# Autodesk Inventor assembly: Roller Piston 4 (.5 and 1 in Stroke, 9-16 in Bore)
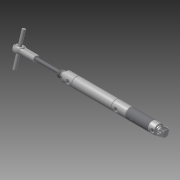
[picture p0: Inventor's stored thumbnail of the model, 180x180]
Saved by Autodesk Inventor 2014 (Build 180170000, 170)
## iProperties
Category: PARTsolutions
Company: BIMBA
Created: 2014-01-20
Part Number: Roller Piston 4 (.5 and 1 in Stroke, 9-16 in Bore)
Catalog Web Link: www.cadenas.de
Description: Original Line Three-Position Cylinders-
Vendor: BIMBA
Document SubType Name: Assembly
Designer: Michael
Manufacturer: BIMBA
PSOL_IDENT_0: {$CADENAS_DATA\23d-libs\bimba\bimba\bimba_imperial\bimba_full_line\original_line_cylinders\three_pos
PSOL_IDENT_1: ition_cylinders\3position_asmtab.prj},283 {VTYP=3D},{STYP=ASSTAB},{NB=020.5/1-DXP(D-12321-A)},{LINA=
PSOL_IDENT_2: 020.5/1-DXP},{NN=Original Line Three-Position Cylinders},{DATE=15.10.2013 05:44:09},{GEOMDATE=27.08.
PSOL_IDENT_3: 2012},{VERSION=},{LINEID=40},{LINESUBID=-1},{WBVAR=STROKEA,STROKEB,MNT,NR,M,NT,EE,EEL,G,K,Q,B,T,W,T1
PSOL_IDENT_4: ,T2,T3,T4,PRC,MB,MN,PB}  {NB=020.5/1-DXP(D-12321-A)},{LINA=020.5/1-DXP},{KT=DUMMY},{PN=020.5/1-DXP},
PSOL_IDENT_5: {PNC=020.5/1-DXP(D-12321-A)},{PNA=(D-12321-A)},{DASH=-},{BORE1=0.56250000},{BORE=9/16\" (02)},{BOREP
PSOL_IDENT_6: N=02},{STROKEA=0.500},{STROKEB=1.000},{STROKEALGA=[0.011:31.989/0.001]},{STROKEALGB=[0.011:31.5/0.00
PSOL_IDENT_7: 1]},{STROKEBMAX=31.5},{STROKE1=0.5},{STROKE2=1.000},{AC=Double Acting},{ACTING=D},{ACTINGALG= 'D' , '
PSOL_IDENT_8: Double Acting' },{ACTINGPN=D},{MNT=XP},{MNTALG= '' , 'Nose Mounting (3P)' , 'XP' , 'Universal Mounti
PSOL_IDENT_9: ng (3P)' },{MNTPN=XP},{TYPE=},{NR=},{NRALG= '' , 'Round (Standard)' , 'NR' , 'Non-Rotating Square' }
PSOL_IDENT_10: ,{NRPN=},{M=},{MALG= '', 'Without Magnet', 'M', 'With Magnet' },{MATR=303 Stainless Steel},{F=},{FAL
PSOL_IDENT_11: G= '', 'Non-Coated (Standard)', 'F', 'Molycoated' },{FPN=},{NT=},{NTPN=},{EE=},{EEL=0.000},{EEMAX=30
PSOL_IDENT_12: .500},{EEALG= '', 'Without Extra Extension', 'EE', 'With Extra Extension' },{EELALG=0},{EEPN=},{EEPN
PSOL_IDENT_13: 1=0.000},{G=},{GPN=},{GPN1=},{K=},{KALG= '', 'Standard' , 'K' , 'Ports Rotated 90deg K' },{KPN=},{Q=
PSOL_IDENT_14: },{QALG= '' , 'N/A' },{QPN=},{B=},{BALG= '', 'Without Bumper' , 'B' , 'With Bumper' },{BPN=},{T=},{T
PSOL_IDENT_15: ALG= '' , 'Standard -20° to 200°F (-29° to 95°C)' , 'N' , 'Low Temperature' , 'V' , 'High Temperatur
PSOL_IDENT_16: e' },{NPN=},{VPN=},{W=},{WALG= '' , 'Without Wiper' , 'W' , 'With Wiper' },{WPN=},{E=},{EALG= '' , '
PSOL_IDENT_17: Standard Seals/Lube' , 'E' , 'Non-Lube Seals/Lube' },{EPN=},{ST=},{STALG= '' , 'Without Switch Track'
PSOL_IDENT_18: , '-' , 'With Switch Track' },{STPALG= '' , 'N/A' },{STPN=},{T1=},{T2=},{T3=},{T4=},{S=},{SALG='','
PSOL_IDENT_19: N/A'},{SPN=},{PRC=},{PRCALG= '' , 'w/out Pivot Rod Clevis' , 'D-850' , 'D-850'},{PRCPN=},{MB=},{MN=}
PSOL_IDENT_20: ,{PB=D-12321-A},{PBALG= '' , 'w/out Pivot Bracket' , 'D-12321-A' , 'D-12321-A' },{PBPN=(D-12321-A)},
PSOL_IDENT_21: {TLEN=2.007},{TEXT=0.133333},{SPACE=0.07619},{FRAC=4.47},{BL=},{BR=},{DWGC=},{PNN=},{MNTRG=},{ACTING
PSOL_IDENT_22: RG=R},{DIMBRL=2.28100000},{DIMBRE=1.65600000},{DIMBBL=1.00000000},{RLB=3.781},{REB=3.156},{BLB=2.500
PSOL_IDENT_23: },{DIMARL=1.85600000},{DIMARE=1.23100000},{DIMABL=0.93800000},{RLA=2.356},{REA=1.731},{BLA=1.438},{D
PSOL_IDENT_24: WGCS=D-68355},{DWGTA=D-75938},{DWGTB=D-7516},{DWGRH=D-15705},{DWGRG=D-26368},{TRANS=0.50000000},{DWG
PSOL_IDENT_25: RCB=D-7508},{DWGRCA=D-9538},{BRL=2.50000000},{BRE=1.57800000},{BBL=1.06200000},{ARL=1.91600000},{ARE=
PSOL_IDENT_26: 0.99400000},{ABL=1.06200000},{T1ALG='','N/A'},{T2ALG='','N/A'},{T3ALG='','N/A'},{T4ALG='','N/A'},{DW
PSOL_IDENT_27: GST=D-74168},{DWGS=},{STL=2.15},{TS=X},{SS=},{AA=4.40},{BA=2.25},{C=0.75},{D=#10-32},{E1=0.38},{E11=
PSOL_IDENT_28: 0.38000000},{E12=0.38000000},{F1=0.06},{G1=N/A},{H=0.50},{I=7/16-20},{J=N/A},{K1=#10-32},{L1=.434/.4
PSOL_IDENT_29: 37},{M1=0.38},{N=0.31},{O=0.62},{AA1=4.12000000},{BA1=2.25000000},{AA1B=4.31000000},{BA1B=2.31000000
PSOL_IDENT_30: },{AA1XP=4.40000000},{BA1XP=2.25000000},{AA1BXP=4.59000000},{BA1BXP=2.31000000},{M11=0.19000000},{M1
PSOL_IDENT_31: 2=0.38000000},{N1=0.50000000},{N2=0.31000000},{O1=0.62000000},{O2=0.62000000},{P=0.25},{Q1=0.19},{R=
PSOL_IDENT_32: 0.16},{P1=0.25000000},{Q11=0.19000000},{R1=0.16},{MBALG= '' , 'w/out Mounting Bracket' , 'F,D-770' ,
PSOL_IDENT_33: 'D-770 (front)', 'R,D-770' , 'D-770 (rear)', '2x,D-770' , 'D-770 (front & rear)' },{MBPN=},{MBP=},{
PSOL_IDENT_34: MNALG= '' , 'w/out Mounting Nut' , 'F,D-154' , 'D-154 (front)', 'R,D-154' , 'D-154 (rear)', '2x,D-15
PSOL_IDENT_35: 4' , 'D-154 (front & rear)' },{MNPN=},{MNP=},{PRCP=},{MBR=},{MBF=},{MNF=},{MNR=},{PBPNALL=D-12321-A}
PSOL_IDENT_36: ,{MBPNALL=D-770},{PRCPNALL=D-850},{FNUTPN=D-154},{RNUTPN=D-154},{ASSOPTACC=T4},{MATALGHTML=<b>Origin
PSOL_IDENT_37: al Line Three Position:</b><dl><dt>Rod:</dt><dd>- 303 Stainless Steel</dd><dt>Bearings:</dt><dd>- Si
PSOL_IDENT_38: ntered Bronze</dd><dt>Body:</dt><dd>- 304 Stainless Steel</dd><dt>End Caps:</dt><dd>- Aluminum</dd><
PSOL_IDENT_39: dt>Seals:</dt><dd>-  Buna N</dd></dl>},{PPATH=three_pos_cylinder_asmtpl.prj}
CNS_NN: Original Line Three-Position Cylinders
CNS_NT: Standard Male Thread
CNS_NB: 020.5/1-DXP(D-12321-A)
CNS_NBSYN: $PNC.
CNS_LINA: 020.5/1-DXP
CNS_PN: 020.5/1-DXP
CNS_PNC: 020.5/1-DXP(D-12321-A)
CNS_PNA: (D-12321-A)
CNS_DASH: -
CNS_BORE1: 0.56250000
CNS_BORE: 9/16" [02]
CNS_BOREPN: 02
CNS_STROKEA: 0.500
CNS_STROKEB: 1.000
CNS_STROKEALGA: [0.011:31.989/0.001]
CNS_STROKEALGB: [0.011:31.5/0.001]
CNS_STROKEBMAX: 31.500
CNS_STROKE1: 0.500
CNS_STROKE2: 1.000
CNS_AC: Double
CNS_ACTING: D
CNS_ACTINGALG: 'D' , 'Double Acting'
CNS_ACTINGPN: D
CNS_MNT: Universal Double End or Rear Pivot [DXP]
CNS_MNTALG: '' , 'Nose Mounting (3P)' , 'XP' , 'Universal Mounting (3P)'
CNS_MNTPN: XP
CNS_NR: Standard Round
CNS_NRALG: '' , 'Round (Standard)' , 'NR' , 'Non-Rotating Square'
CNS_M: Without Magnet Piston
CNS_MALG: '', 'Without Magnet', 'M', 'With Magnet'
CNS_MATR: Stainless Steel
CNS_FALG: '', 'Non-Coated (Standard)', 'F', 'Molycoated'
CNS_EE: Standard Rod Extension
CNS_EEL: 0.000
CNS_EEMAX: 30.500
CNS_EEALG: '', 'Without Extra Extension', 'EE', 'With Extra Extension'
CNS_EELALG: 0
CNS_EEPN1: 0.000
CNS_G: Standard Grease Lube
CNS_K: Standard
CNS_KALG: '', 'Standard' , 'K' , 'Ports Rotated 90deg K'
CNS_Q: N/A
CNS_QALG: '' , 'N/A'
CNS_B: Without Bumpers
CNS_BALG: '', 'Without Bumper' , 'B' , 'With Bumper'
CNS_T: Standard -20° to 200°F (-29° to 95°C)
CNS_TALG: '' , 'Standard -20° to 200°F (-29° to 95°C)' , 'N' , 'Low Temperature' , 'V' , 'High Temperature'
CNS_W: Without Wiper
CNS_WALG: '' , 'Without Wiper' , 'W' , 'With Wiper'
CNS_EALG: '' , 'Standard Seals/Lube' , 'E' , 'Non-Lube Seals/Lube'
CNS_STALG: '' , 'Without Switch Track' , '-' , 'With Switch Track'
CNS_STPALG: '' , 'N/A'
CNS_T1: N/A
CNS_T2: N/A
CNS_T3: N/A
CNS_T4: N/A
CNS_SALG: '','N/A'
CNS_PRC: Without Piston Rod Clevis
CNS_PRCALG: '' , 'w/out Pivot Rod Clevis' , 'D-850' , 'D-850'
CNS_MB: Without Mounting Bracket
CNS_MN: Without Mounting Nut
CNS_PB: D-12321-A
CNS_PBALG: '' , 'w/out Pivot Bracket' , 'D-12321-A' , 'D-12321-A'
CNS_PBPN: (D-12321-A)
CNS_TLEN: 2.007
CNS_TEXT: 0.133
CNS_SPACE: 0.076
CNS_FRAC: 4.470
CNS_ACTINGRG: R
CNS_DIMBRL: 2.28100000
CNS_DIMBRE: 1.65600000
CNS_DIMBBL: 1.00000000
CNS_RLB: 3.781
CNS_REB: 3.156
CNS_BLB: 2.500
CNS_DIMARL: 1.85600000
CNS_DIMARE: 1.23100000
CNS_DIMABL: 0.93800000
CNS_RLA: 2.356
CNS_REA: 1.731
CNS_BLA: 1.438
CNS_DWGCS: D-68355
CNS_DWGTA: D-75938
CNS_DWGTB: D-7516
CNS_DWGRH: D-15705
CNS_DWGRG: D-26368
CNS_TRANS: 0.50000000
CNS_DWGRCB: D-7508
CNS_DWGRCA: D-9538
CNS_BRL: 2.50000000
CNS_BRE: 1.57800000
CNS_BBL: 1.06200000
CNS_ARL: 1.91600000
CNS_ARE: 0.99400000
CNS_ABL: 1.06200000
CNS_T1ALG: '','N/A'
CNS_T2ALG: '','N/A'
CNS_T3ALG: '','N/A'
CNS_T4ALG: '','N/A'
CNS_DWGST: D-74168
CNS_STL: 2.150
CNS_TS: X
CNS_AA: 4.40
CNS_BA: 2.25
CNS_C: 0.75
CNS_D: #10-32
CNS_E1: 0.38
CNS_E11: 0.38000000
CNS_E12: 0.38000000
CNS_F1: 0.06
CNS_G1: N/A
CNS_H: 0.50
CNS_I: 7/16-20
CNS_J: N/A
CNS_K1: #10-32
CNS_L1: .434/.437
CNS_M1: 0.38
CNS_N: 0.31
CNS_O: 0.62
CNS_AA1: 4.12000000
CNS_BA1: 2.25000000
CNS_AA1B: 4.31000000
CNS_BA1B: 2.31000000
CNS_AA1XP: 4.40000000
CNS_BA1XP: 2.25000000
CNS_AA1BXP: 4.59000000
CNS_BA1BXP: 2.31000000
CNS_M11: 0.19000000
CNS_M12: 0.38000000
CNS_N1: 0.50000000
CNS_N2: 0.31000000
CNS_O1: 0.62000000
CNS_O2: 0.62000000
CNS_P: 0.25
CNS_Q1: 0.19
CNS_R: 0.16
CNS_P1: 0.25000000
CNS_Q11: 0.19000000
CNS_R1: 0.16
CNS_MBALG: '' , 'w/out Mounting Bracket' , 'F,D-770' , 'D-770 (front)', 'R,D-770' , 'D-770 (rear)', '2x,D-770' , 'D-770 (front & rear)'
CNS_MNALG: '' , 'w/out Mounting Nut' , 'F,D-154' , 'D-154 (front)', 'R,D-154' , 'D-154 (rear)', '2x,D-154' , 'D-154 (front & rear)'
CNS_PBPNALL: D-12321-A
CNS_MBPNALL: D-770
CNS_PRCPNALL: D-850
CNS_FNUTPN: D-154
CNS_RNUTPN: D-154
CNS_ASSOPTACC: T4
CNS_MATALGHTML: <b>Original Line Three Position:</b><dl><dt>Rod:</dt><dd>- 303 Stainless Steel</dd><dt>Bearings:</dt><dd>- Sintered Bronze</dd><dt>Body:</dt><dd>- 304 Stainless Steel</dd><dt>End Caps:</dt><dd>- Aluminum</dd><dt>Seals:</dt><dd>-  Buna N</dd></dl>
CNS_PPATH: three_pos_cylinder_asmtpl.prj
SUPPLIER: BIMBA
ARTICLENO: 020.5/1-DXP(D-12321-A)
BOMINFO: 020.5/1-DXP
CREATOR: CADENAS GmbH
Title: 020.5/1-DXP
Author: Cadenas PARTsolutions
## Documents named in this file (15)
- C:\Users\Michael\Documents\GitHub\2014buildCAD\Duluth Collector\Roller Piston 4 (.5 and 1 in Stroke, 9-16 in Bore).iam
- C:\Users\Michael\Documents\GitHub\2014buildCAD\New Collector\020_5_1-DXP(D-12321-A)0_dummy.ipt
- C:\Users\Michael\Documents\GitHub\2014buildCAD\New Collector\D-68355-XP--0.ipt
- C:\Users\Michael\Documents\GitHub\2014buildCAD\New Collector\D-75938XP-1_438.ipt
- C:\Users\Michael\Documents\GitHub\2014buildCAD\New Collector\D-15705rear_head.ipt
- C:\Users\Michael\Documents\GitHub\2014buildCAD\New Collector\D-8597.ipt
- C:\Users\Michael\Documents\GitHub\2014buildCAD\New Collector\D-12321-A-dummy.ipt
- C:\Users\Michael\Documents\GitHub\2014buildCAD\New Collector\D-9769-clevis_pin.ipt
- C:\Users\Michael\Documents\GitHub\2014buildCAD\New Collector\D-9770-rr.ipt
- C:\Users\Michael\Documents\GitHub\2014buildCAD\New Collector\D-7516XP-2_5.ipt
- C:\Users\Michael\Documents\GitHub\2014buildCAD\New Collector\D-26368----0_5_rod_guide_cyl.ipt
- C:\Users\Michael\Documents\GitHub\2014buildCAD\New Collector\D-75080_5-1XP-3_781-3pos.ipt
- C:\Users\Michael\Documents\GitHub\2014buildCAD\New Collector\D-95380_5-1XP-2_356-3pos.ipt
- C:\Users\Michael\Documents\GitHub\2014buildCAD\New Collector\Axle 0.190 in 3 in length.ipt
- C:\Users\Michael\Documents\GitHub\2014buildCAD\New Collector\Rod End (McMaster Part #6498K592).ipt
## Components (15 placed, 14 different names)
1. 020_5_1-DXP(D-12321-A)0_dummy:1 — dummy_XY@1 <-> centar_XY@2, dummy_Z@1 <-> centar_Z@2, dummy_YZ@1 <-> centar_YZ@2
2. D-68355-XP--0:1 — dummy_XY@1 <-> centar_XY@2, dummy_Z@1 <-> centar_Z@2, dummy_YZ@1 <-> centar_YZ@2, to_cyl_A_XY@2 <-> tube2_XY@3, to_cyl_A_Z@2 <-> tube2_Z@3, to_cyl_A_YZ@2 <-> tube2_YZ@3, to_cyl_B_XY@2 <-> tube1_XY@12, to_cyl_B_Z@2 <-> tube1_Z@12, to_cyl_B_YZ@2 <-> tube1_YZ@12, to_rod_A_XY@2 <-> to_rod_guide_XY@15, to_rod_A_Z@2 <-> to_rod_guide_Z@15
3. D-75938XP-1_438:1 — to_cyl_A_XY@2 <-> tube2_XY@3, to_cyl_A_Z@2 <-> tube2_Z@3, to_cyl_A_YZ@2 <-> tube2_YZ@3, tube1_XY@3 <-> rear_head_XY@4, tube1_Z@3 <-> rear_head_Z@4, tube1_YZ@3 <-> rear_head_YZ@4
4. D-15705rear_head:1 — tube1_XY@3 <-> rear_head_XY@4, tube1_Z@3 <-> rear_head_Z@4, tube1_YZ@3 <-> rear_head_YZ@4, to_bushing_XY@4 <-> bushing_XY@5, to_bushing_Z@4 <-> bushing_Z@5, to_bushing_YZ@4 <-> bushing_YZ@5, to_pivot_bracket_XY@4 <-> to_cyl_XY@6, to_pivot_bracket_Z@4 <-> to_cyl_Z@6, Mate:33
5. D-8597:1 — to_bushing_XY@4 <-> bushing_XY@5, to_bushing_Z@4 <-> bushing_Z@5, to_bushing_YZ@4 <-> bushing_YZ@5, Mate:32
6. D-12321-A-dummy:1 — to_pivot_bracket_XY@4 <-> to_cyl_XY@6, to_pivot_bracket_Z@4 <-> to_cyl_Z@6
7. D-9769-clevis_pin:1 — rr1_XY@9 <-> rr_XY@10, rr1_Z@9 <-> rr_Z@10, rr1_YZ@9 <-> rr_YZ@10, rr2_XY@9 <-> rr_XY@11, rr2_Z@9 <-> rr_Z@11, rr2_YZ@9 <-> rr_YZ@11, Mate:32
8. D-9770-rr:1 — rr1_XY@9 <-> rr_XY@10, rr1_Z@9 <-> rr_Z@10, rr1_YZ@9 <-> rr_YZ@10, Mate:33
9. D-9770-rr:2 — rr2_XY@9 <-> rr_XY@11, rr2_Z@9 <-> rr_Z@11, rr2_YZ@9 <-> rr_YZ@11
10. D-7516XP-2_5:1 — to_cyl_B_XY@2 <-> tube1_XY@12, to_cyl_B_Z@2 <-> tube1_Z@12, to_cyl_B_YZ@2 <-> tube1_YZ@12, tube2_XY@12 <-> to_tube_XY@13, tube2_Z@12 <-> to_tube_Z@13, tube2_YZ@12 <-> to_tube_YZ@13
11. D-26368----0_5_rod_guide_cyl:1 — tube2_XY@12 <-> to_tube_XY@13, tube2_Z@12 <-> to_tube_Z@13, tube2_YZ@12 <-> to_tube_YZ@13, to_rod_XY@13 <-> to_rod_guide_XY@14, to_rod_Z@13 <-> to_rod_guide_Z@14
12. D-75080_5-1XP-3_781-3pos:1 — to_rod_XY@13 <-> to_rod_guide_XY@14, to_rod_Z@13 <-> to_rod_guide_Z@14, Mate:24, Mate:30
13. D-95380_5-1XP-2_356-3pos:1 — to_rod_A_XY@2 <-> to_rod_guide_XY@15, to_rod_A_Z@2 <-> to_rod_guide_Z@15
14. Axle 0.190 in 3 in length:1 — Mate:26, Flush:6
15. Rod End (McMaster Part #6498K592):1 — Mate:24, Mate:26, Flush:6, Mate:30
## Relationships (36: Mate 24, Angle 8, Flush 4)
- dummy_XY@1 <-> centar_XY@2 [Mate]: 020_5_1-DXP(D-12321-A)0_dummy:1 ↔ D-68355-XP--0:1
- dummy_Z@1 <-> centar_Z@2 [Mate]: 020_5_1-DXP(D-12321-A)0_dummy:1 ↔ D-68355-XP--0:1
- dummy_YZ@1 <-> centar_YZ@2 [Angle] (-90 deg): 020_5_1-DXP(D-12321-A)0_dummy:1 ↔ D-68355-XP--0:1
- to_cyl_A_XY@2 <-> tube2_XY@3 [Flush]: D-68355-XP--0:1 ↔ D-75938XP-1_438:1
- to_cyl_A_Z@2 <-> tube2_Z@3 [Mate]: D-68355-XP--0:1 ↔ D-75938XP-1_438:1
- to_cyl_A_YZ@2 <-> tube2_YZ@3 [Angle] (0 deg): D-68355-XP--0:1 ↔ D-75938XP-1_438:1
- tube1_XY@3 <-> rear_head_XY@4 [Mate]: D-75938XP-1_438:1 ↔ D-15705rear_head:1
- tube1_Z@3 <-> rear_head_Z@4 [Mate]: D-75938XP-1_438:1 ↔ D-15705rear_head:1
- tube1_YZ@3 <-> rear_head_YZ@4 [Angle] (90 deg): D-75938XP-1_438:1 ↔ D-15705rear_head:1
- to_bushing_XY@4 <-> bushing_XY@5 [Mate]: D-15705rear_head:1 ↔ D-8597:1
- to_bushing_Z@4 <-> bushing_Z@5 [Mate]: D-15705rear_head:1 ↔ D-8597:1
- to_bushing_YZ@4 <-> bushing_YZ@5 [Angle] (0 deg): D-15705rear_head:1 ↔ D-8597:1
- to_pivot_bracket_XY@4 <-> to_cyl_XY@6 [Mate]: D-15705rear_head:1 ↔ D-12321-A-dummy:1
- to_pivot_bracket_Z@4 <-> to_cyl_Z@6 [Mate]: D-15705rear_head:1 ↔ D-12321-A-dummy:1
- rr1_XY@9 <-> rr_XY@10 [Mate]: D-9769-clevis_pin:1 ↔ D-9770-rr:1
- rr1_Z@9 <-> rr_Z@10 [Mate]: D-9769-clevis_pin:1 ↔ D-9770-rr:1
- rr1_YZ@9 <-> rr_YZ@10 [Angle] (0 deg): D-9769-clevis_pin:1 ↔ D-9770-rr:1
- rr2_XY@9 <-> rr_XY@11 [Mate]: D-9769-clevis_pin:1 ↔ D-9770-rr:2
- rr2_Z@9 <-> rr_Z@11 [Mate]: D-9769-clevis_pin:1 ↔ D-9770-rr:2
- rr2_YZ@9 <-> rr_YZ@11 [Angle] (0 deg): D-9769-clevis_pin:1 ↔ D-9770-rr:2
- to_cyl_B_XY@2 <-> tube1_XY@12 [Flush]: D-68355-XP--0:1 ↔ D-7516XP-2_5:1
- to_cyl_B_Z@2 <-> tube1_Z@12 [Mate]: D-68355-XP--0:1 ↔ D-7516XP-2_5:1
- to_cyl_B_YZ@2 <-> tube1_YZ@12 [Angle] (0 deg): D-68355-XP--0:1 ↔ D-7516XP-2_5:1
- tube2_XY@12 <-> to_tube_XY@13 [Mate]: D-7516XP-2_5:1 ↔ D-26368----0_5_rod_guide_cyl:1
- tube2_Z@12 <-> to_tube_Z@13 [Mate]: D-7516XP-2_5:1 ↔ D-26368----0_5_rod_guide_cyl:1
- tube2_YZ@12 <-> to_tube_YZ@13 [Angle] (-180 deg): D-7516XP-2_5:1 ↔ D-26368----0_5_rod_guide_cyl:1
- to_rod_XY@13 <-> to_rod_guide_XY@14 [Flush]: D-26368----0_5_rod_guide_cyl:1 ↔ D-75080_5-1XP-3_781-3pos:1
- to_rod_Z@13 <-> to_rod_guide_Z@14 [Mate]: D-26368----0_5_rod_guide_cyl:1 ↔ D-75080_5-1XP-3_781-3pos:1
- to_rod_A_XY@2 <-> to_rod_guide_XY@15 [Mate]: D-68355-XP--0:1 ↔ D-95380_5-1XP-2_356-3pos:1
- to_rod_A_Z@2 <-> to_rod_guide_Z@15 [Mate]: D-68355-XP--0:1 ↔ D-95380_5-1XP-2_356-3pos:1
- Mate:24: D-75080_5-1XP-3_781-3pos:1 ↔ Rod End (McMaster Part #6498K592):1
- Mate:26: Axle 0.190 in 3 in length:1 ↔ Rod End (McMaster Part #6498K592):1
- Flush:6 (-21.4376 mm): Axle 0.190 in 3 in length:1 ↔ Rod End (McMaster Part #6498K592):1
- Mate:30: D-75080_5-1XP-3_781-3pos:1 ↔ Rod End (McMaster Part #6498K592):1
- Mate:32: D-8597:1 ↔ D-9769-clevis_pin:1
- Mate:33 (2.1209 mm): D-15705rear_head:1 ↔ D-9770-rr:1
